# Autodesk Inventor assembly: Intake Claw Prototype
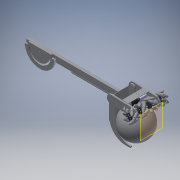
[picture p0: Inventor's stored thumbnail of the model, 180x180]
Saved by Autodesk Inventor 2016 (Build 200138000, 138)
## iProperties
Created: 2016-01-16
Part Number: Intake Claw Prototype
Document SubType Name: Assembly
Designer: Mentor1102
Author: Mentor1102
## Documents named in this file (15)
- C:\Users\Mentor1102\Documents\FRC-4901-Garnet-Squadron\trunk\2016\2016 Robot\Mechanical\4901 Full Inventor CAD\Intake Claw Prototype.iam
- C:\Users\Mentor1102\Documents\FRC-4901-Garnet-Squadron\trunk\2016\2016 Robot\Mechanical\4901 Full Inventor CAD\Top IntakeBar.ipt
- C:\Users\Mentor1102\Documents\FRC-4901-Garnet-Squadron\trunk\2016\2016 Robot\Mechanical\4901 Full Inventor CAD\Bottom IntakeBar.ipt
- C:\Users\Mentor1102\Documents\FRC-4901-Garnet-Squadron\trunk\2016\2016 Robot\Mechanical\4901 Full Inventor CAD\Boulder.ipt
- C:\Users\Mentor1102\Documents\FRC-4901-Garnet-Squadron\trunk\2016\2016 Robot\Mechanical\4901 Full Inventor CAD\Intake Roller.ipt
- C:\Users\Mentor1102\Documents\FRC-4901-Garnet-Squadron\trunk\2016\2016 Robot\Mechanical\4901 Full Inventor CAD\HalfIn Hex Standin.ipt
- C:\Users\Mentor1102\Documents\FRC-4901-Garnet-Squadron\trunk\2016\2016 Robot\Mechanical\4901 Full Inventor CAD\ClawPlate.ipt
- C:\Users\Mentor1102\Documents\FRC-4901-Garnet-Squadron\trunk\2016\2016 Robot\Mechanical\4901 Full Inventor CAD\ArmBar.ipt
- C:\Users\Mentor1102\Documents\FRC-4901-Garnet-Squadron\trunk\2016\2016 Robot\Mechanical\4901 Full Inventor CAD\Pneumatic Cylinder Standin.ipt
- C:\Users\Mentor1102\Documents\FRC-4901-Garnet-Squadron\trunk\2016\2016 Robot\Mechanical\4901 Full Inventor CAD\217-3644-STEP-20151209.iam
- C:\Users\Mentor1102\Documents\FRC-4901-Garnet-Squadron\trunk\2016\2016 Robot\Mechanical\4901 Full Inventor CAD\217-3645-STEP-20151209.iam
- C:\Users\Mentor1102\Documents\FRC-4901-Garnet-Squadron\trunk\2016\2016 Robot\Mechanical\4901 Full Inventor CAD\217-3488-STEP.ipt
- C:\Users\Mentor1102\Documents\FRC-4901-Garnet-Squadron\trunk\2016\2016 Robot\Mechanical\4901 Full Inventor CAD\big_gear.ipt
- C:\Users\Mentor1102\Documents\FRC-4901-Garnet-Squadron\trunk\2016\2016 Robot\Mechanical\4901 Full Inventor CAD\VEXproBAG.ipt
- C:\Users\Mentor1102\Documents\FRC-4901-Garnet-Squadron\trunk\2016\2016 Robot\Mechanical\4901 Full Inventor CAD\VersaPlate.ipt
## Components (21 placed, 14 different names)
1. Top IntakeBar:1 — Insert:18, Insert:20, Mate:18, Angle:3
2. Bottom IntakeBar:1 — Insert:1, Mate:7, Mate:8, Insert:18
3. Bottom IntakeBar:2 — Insert:1, Mate:1, Angle:1, Mate:2, Angle:2, Mate:5, Mate:6, Insert:19
4. Top IntakeBar:2 — Insert:16, Insert:17, Insert:19
5. Boulder:1 — Mate:3, Mate:4
6. HalfIn Hex Standin:1 — Insert:16
7. HalfIn Hex Standin:2 — Insert:6, Insert:7, Insert:11, Insert:12, Insert:13, Insert:14, Insert:15, Insert:17
8. Intake Roller:1 — Insert:6
9. Intake Roller:4 — Insert:7
10. ClawPlate:1 — Mate:5, Mate:6, Mate:7, Mate:8, Mate:12, Mate:15, Mate:16, Flush:2
11. ArmBar:1 — Mate:13, Mate:15, Mate:16, Flush:1, Insert:25, Mate:19
12. Pneumatic Cylinder Standin:1 — Mate:12, Mate:13
13. 217-3644-STEP-20151209:1 [sub-assembly] — Insert:11
14. 217-3645-STEP-20151209:1 [sub-assembly] — Insert:12
15. 217-3644-STEP-20151209:2 [sub-assembly] — Insert:14
16. 217-3645-STEP-20151209:2 [sub-assembly] — Insert:13
17. 217-3488-STEP:1 — Insert:20, Insert:24
18. 217-3488-STEP:2 — Insert:15
19. big_gear:1 — Insert:25, Mate:19
20. VEXproBAG:1 — Insert:24, Angle:3, Insert:26, Insert:27
21. VersaPlate:1 — Insert:26, Insert:27
## Relationships (37: Insert 17, Mate 15, Angle 3, Flush 2)
- Insert:1 (152.4 mm): Bottom IntakeBar:1 ↔ Bottom IntakeBar:2
- Mate:1: Bottom IntakeBar:2
- Angle:1 (0 deg): Bottom IntakeBar:2
- Mate:2: Bottom IntakeBar:2
- Angle:2 (0 deg): Bottom IntakeBar:2
- Mate:3: Boulder:1
- Mate:4: Boulder:1
- Insert:6 (-114.3 mm): HalfIn Hex Standin:2 ↔ Intake Roller:1
- Insert:7 (-114.3 mm): HalfIn Hex Standin:2 ↔ Intake Roller:4
- Mate:5: Bottom IntakeBar:2 ↔ ClawPlate:1
- Mate:6: Bottom IntakeBar:2 ↔ ClawPlate:1
- Mate:7: Bottom IntakeBar:1 ↔ ClawPlate:1
- Mate:8: Bottom IntakeBar:1 ↔ ClawPlate:1
- Mate:12: ClawPlate:1 ↔ Pneumatic Cylinder Standin:1
- Mate:13: ArmBar:1 ↔ Pneumatic Cylinder Standin:1
- Insert:11 (-165.1 mm): HalfIn Hex Standin:2 ↔ 217-3644-STEP-20151209:1
- Insert:12 (-165.1 mm): HalfIn Hex Standin:2 ↔ 217-3645-STEP-20151209:1
- Insert:13 (-76.2 mm): HalfIn Hex Standin:2 ↔ 217-3645-STEP-20151209:2
- Insert:14 (-76.2 mm): HalfIn Hex Standin:2 ↔ 217-3644-STEP-20151209:2
- Insert:15 (-99.06 mm): HalfIn Hex Standin:2 ↔ 217-3488-STEP:2
- Insert:16 (-279.4 mm): Top IntakeBar:2 ↔ HalfIn Hex Standin:1
- Insert:17 (-279.4 mm): Top IntakeBar:2 ↔ HalfIn Hex Standin:2
- Insert:18: Top IntakeBar:1 ↔ Bottom IntakeBar:1
- Insert:19: Bottom IntakeBar:2 ↔ Top IntakeBar:2
- Insert:20 (-22.86 mm): Top IntakeBar:1 ↔ 217-3488-STEP:1
- Insert:24: 217-3488-STEP:1 ↔ VEXproBAG:1
- Mate:15: ClawPlate:1 ↔ ArmBar:1
- Mate:16: ClawPlate:1 ↔ ArmBar:1
- Flush:1 (-12.7 mm): ArmBar:1
- Mate:17
- Mate:18 (88.9 mm): Top IntakeBar:1
- Insert:25: ArmBar:1 ↔ big_gear:1
- Mate:19: ArmBar:1 ↔ big_gear:1
- Flush:2 (275.59 mm): ClawPlate:1
- Angle:3 (90 deg): Top IntakeBar:1 ↔ VEXproBAG:1
- Insert:26 (17.018 mm): VEXproBAG:1 ↔ VersaPlate:1
- Insert:27 (17.018 mm): VEXproBAG:1 ↔ VersaPlate:1
